# Autodesk Inventor assembly: PiWithCase-SubAssembly
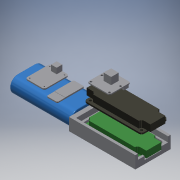
[picture p0: Inventor's stored thumbnail of the model, 180x180]
Saved by Autodesk Inventor 2019 (Build 230136000, 136)
## iProperties
Created: 2019-04-12
Part Number: PiWithCase-SubAssembly
Document SubType Name: Assembly
Designer: Epsilon
Author: Epsilon
## Documents named in this file (8)
- F:\Code\3D-Scanner-Hardware\Assembly\PiWithCase-SubAssembly.iam
- F:\Code\3D-Scanner-Hardware\PiHolder.ipt
- F:\Code\3D-Scanner-Hardware\ExistingParts\RaspberryPi0W-SafeSpecs.ipt
- F:\Code\3D-Scanner-Hardware\ExistingParts\4400mAh-LiIon-Battery.ipt
- F:\Code\3D-Scanner-Hardware\ExistingParts\Adafruit-PowerBoost500.ipt
- F:\Code\3D-Scanner-Hardware\ExistingParts\RaspberryPi0W-BerryIMUV3-SafeSpecs.ipt
- F:\Code\3D-Scanner-Hardware\ExistingParts\RaspberryPiCamera.ipt
- F:\Code\3D-Scanner-Hardware\ExistingParts\Adafruit-MicroLipoBatteryCharger.ipt
## Components (7 placed, 7 different names)
1. PiHolder:1 — Mate:1, Mate:2, Mate:3, Mate:4
2. RaspberryPi0W-SafeSpecs:1 — Mate:1, Mate:2, Mate:3
3. 4400mAh-LiIon-Battery:1 — Mate:4
4. Adafruit-PowerBoost500:1
5. RaspberryPi0W-BerryIMUV3-SafeSpecs:1
6. RaspberryPiCamera:1
7. Adafruit-MicroLipoBatteryCharger:1
## Relationships (4: Mate 4)
- Mate:1: PiHolder:1 ↔ RaspberryPi0W-SafeSpecs:1
- Mate:2: PiHolder:1 ↔ RaspberryPi0W-SafeSpecs:1
- Mate:3: PiHolder:1 ↔ RaspberryPi0W-SafeSpecs:1
- Mate:4: PiHolder:1 ↔ 4400mAh-LiIon-Battery:1
